# Autodesk Inventor assembly: WaterproofCoverNRotatingPart
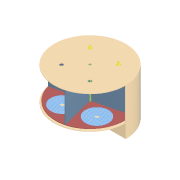
[picture p0: Inventor's stored thumbnail of the model, 180x180]
Saved by Autodesk Inventor 2018 (Build 220112000, 112)
## iProperties
Created: 2017-12-09
Part Number: WaterproofCoverNRotatingPart
Document SubType Name: Assembly
Designer: Udara Wanasinghe
Author: Udara Wanasinghe
## Documents named in this file (4)
- D:\Documents\FIT\Hardware Project\Perfect\WaterproofCoverNRotatingPart.iam
- D:\Documents\FIT\Hardware Project\Perfect\RotatingPart.iam
- D:\Documents\FIT\Hardware Project\Perfect\WaterproofCover.ipt
- D:\Documents\FIT\Hardware Project\Perfect\Nozzle.ipt
## Components (6 placed, 3 different names)
1. WaterproofCover:1 — Rotational:1, Rigid:1, Rigid:2, Rigid:3, Rotational:2
2. RotatingPart:1 [sub-assembly] — Rotational:1
3. Nozzle:1 — Rigid:1
4. Nozzle:2 — Rigid:2
5. Nozzle:3 — Rotational:2
6. Nozzle:4 — Rigid:3
## Relationships (5: WeldJoint 3, RevoluteJoint 2)
- Rotational:1 [RevoluteJoint]: WaterproofCover:1 ↔ RotatingPart:1
- Rigid:1 [WeldJoint]: WaterproofCover:1 ↔ Nozzle:1
- Rigid:2 [WeldJoint]: WaterproofCover:1 ↔ Nozzle:2
- Rigid:3 [WeldJoint]: WaterproofCover:1 ↔ Nozzle:4
- Rotational:2 [RevoluteJoint]: WaterproofCover:1 ↔ Nozzle:3
